# Autodesk Inventor assembly: tandembox_intivo
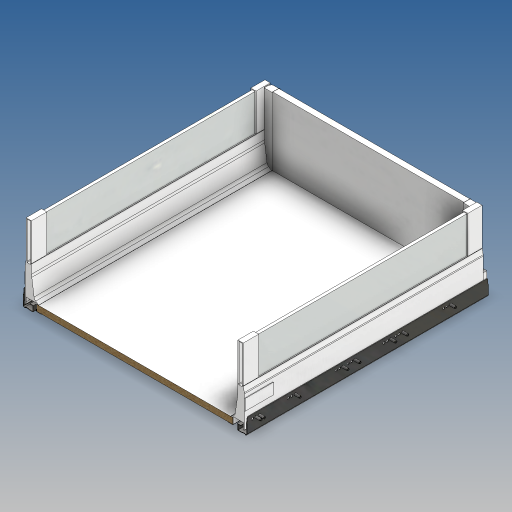
[picture p0: Inventor's stored thumbnail of the model, 512x512]
Saved by Autodesk Inventor 2023 (Build 270158000, 158)
## iProperties
RuleStatus: InUse
Category: Drawer
AfterAnyParamChange0: ConstraintRule
AfterComponentSuppressionChange0: ConstraintRule
Created: 2020-01-10
Part Number: tandembox_intivo
Document SubType Name: Assembly
Designer: RokasM
Author: RokasM
## iProperties of the stored document MemberDocs/xAaaaavdaAaaaaaaaAaaaq5iiOc
Category: Drawer
RuleStatus: InUse
Created: 2020-01-10
Part Number: tandembox_intivo
Document SubType Name: Assembly
Designer: RokasM
AfterAnyParamChange0: ConstraintRule
AfterComponentSuppressionChange0: ConstraintRule
Author: RokasM
## Documents named in this file (41)
- C:\W4INV 2024 Design\iBOX LIBRARY\Drawers\Blum TANDEMBOX\tandembox_intivo.iam
- @tandembox_intivo.iam
- C:\W4INV 2023 Design\iBOX LIBRARY\Drawers\Blum TANDEMBOX\Parts\01_base.ipt
- C:\W4INV 2023 Design\iBOX LIBRARY\Drawers\Blum TANDEMBOX\Parts\02_back.ipt
- C:\W4INV 2023 Design\iBOX LIBRARY\Drawers\Blum TANDEMBOX\Parts\03_drawer_side.ipt
- C:\W4INV 2023 Design\iBOX LIBRARY\Drawers\Blum TANDEMBOX\Parts\04_right_fixing.ipt
- C:\W4INV 2023 Design\iBOX LIBRARY\Drawers\Blum TANDEMBOX\Parts\05_boxcover_front.ipt
- C:\W4INV 2023 Design\iBOX LIBRARY\Drawers\Blum TANDEMBOX\Parts\06_boxcover_back.ipt
- C:\W4INV 2023 Design\iBOX LIBRARY\Drawers\Blum TANDEMBOX\Parts\07_cabinet_profile.ipt
- C:\W4INV 2023 Design\iBOX LIBRARY\Drawers\Blum TANDEMBOX\Parts\08_roller.ipt
- C:\W4INV 2023 Design\iBOX LIBRARY\Drawers\Blum TANDEMBOX\Parts\09_glass.ipt
- C:\W4INV 2023 Design\iBOX LIBRARY\Drawers\Blum TANDEMBOX\Parts\10_hole1.ipt
- C:\W4INV 2023 Design\iBOX LIBRARY\Drawers\Blum TANDEMBOX\Parts\11_hole2.ipt
- C:\W4INV 2023 Design\iBOX LIBRARY\Drawers\Blum TANDEMBOX\Parts\12_hole3.ipt
- C:\W4INV 2023 Design\iBOX LIBRARY\Drawers\Blum TANDEMBOX\Parts\13_hole4.ipt
- C:\W4INV 2023 Design\iBOX LIBRARY\Drawers\Blum TANDEMBOX\Parts\14_hole5.ipt
- C:\W4INV 2023 Design\iBOX LIBRARY\Drawers\Blum TANDEMBOX\Parts\15_hole6.ipt
- C:\W4INV 2023 Design\iBOX LIBRARY\Drawers\Blum TANDEMBOX\Parts\16_hole7.ipt
- C:\W4INV 2023 Design\iBOX LIBRARY\Drawers\Blum TANDEMBOX\Parts\17_screw.ipt
- C:\W4INV 2023 Design\iBOX LIBRARY\Drawers\Blum TANDEMBOX\tandembox_intivo.ipt
- C:\W4INV 2023 Design\iBOX LIBRARY\Drawers\Blum TANDEMBOX\Parts\18_boxcap.ipt
- C:\W4INV 2024 Design\iBOX LIBRARY\Drawers\Blum TANDEMBOX\Parts\01_base.ipt
- C:\W4INV 2024 Design\iBOX LIBRARY\Drawers\Blum TANDEMBOX\Parts\02_back.ipt
- C:\W4INV 2024 Design\iBOX LIBRARY\Drawers\Blum TANDEMBOX\Parts\03_drawer_side.ipt
- C:\W4INV 2024 Design\iBOX LIBRARY\Drawers\Blum TANDEMBOX\Parts\04_right_fixing.ipt
- C:\W4INV 2024 Design\iBOX LIBRARY\Drawers\Blum TANDEMBOX\Parts\05_boxcover_front.ipt
- C:\W4INV 2024 Design\iBOX LIBRARY\Drawers\Blum TANDEMBOX\Parts\06_boxcover_back.ipt
- C:\W4INV 2024 Design\iBOX LIBRARY\Drawers\Blum TANDEMBOX\Parts\07_cabinet_profile.ipt
- C:\W4INV 2024 Design\iBOX LIBRARY\Drawers\Blum TANDEMBOX\Parts\08_roller.ipt
- C:\W4INV 2024 Design\iBOX LIBRARY\Drawers\Blum TANDEMBOX\Parts\09_glass.ipt
- C:\W4INV 2024 Design\iBOX LIBRARY\Drawers\Blum TANDEMBOX\Parts\10_hole1.ipt
- C:\W4INV 2024 Design\iBOX LIBRARY\Drawers\Blum TANDEMBOX\Parts\11_hole2.ipt
- C:\W4INV 2024 Design\iBOX LIBRARY\Drawers\Blum TANDEMBOX\Parts\12_hole3.ipt
- C:\W4INV 2024 Design\iBOX LIBRARY\Drawers\Blum TANDEMBOX\Parts\13_hole4.ipt
- C:\W4INV 2024 Design\iBOX LIBRARY\Drawers\Blum TANDEMBOX\Parts\14_hole5.ipt
- C:\W4INV 2024 Design\iBOX LIBRARY\Drawers\Blum TANDEMBOX\Parts\15_hole6.ipt
- C:\W4INV 2024 Design\iBOX LIBRARY\Drawers\Blum TANDEMBOX\Parts\16_hole7.ipt
- C:\W4INV 2024 Design\iBOX LIBRARY\Drawers\Blum TANDEMBOX\Parts\17_screw.ipt
- C:\W4INV 2024 Design\iBOX LIBRARY\Drawers\Blum TANDEMBOX\tandembox_intivo.ipt
- C:\W4INV 2024 Design\iBOX LIBRARY\Drawers\Blum TANDEMBOX\Parts\18_boxcap.ipt
- C:\W4INV 2023 Design\iBOX LIBRARY\Drawers\Blum TANDEMBOX\tandembox_intivo.iam
## Components (26 placed, 19 different names)
1. @skeleton
2. @01_base:1 — Flush:14, Flush:15, Flush:16
3. @02_back:1 — Flush:9, Flush:10, Flush:11, Flush:23, Flush:24
4. @03_drawer_side:1 — Flush:1, Mate:8, Flush:2, Flush:3, Mate:9, Mate:10, Flush:12, Flush:13, Flush:14, Flush:15, Flush:16, Flush:17, Flush:21, Mate:12, Flush:22
5. @04_right_fixing:1 — Flush:6, Flush:7, Flush:8, Flush:9, Flush:10, Flush:11, Flush:25
6. @05_boxcover_front:1 — Flush:1, Mate:8, Flush:2, Flush:4, Flush:5, Mate:11
7. @06_boxcover_back:1 — Flush:3, Mate:9, Mate:10, Flush:6, Flush:7, Flush:8
8. @07_cabinet_profile:1 — Flush:12, Flush:13, Flush:18, Flush:19, Flush:20, Flush:26, Flush:27, Flush:28, Flush:29, Mate:13, Mate:14, Mate:15, Mate:16, Flush:30, Mate:17
9. @08_roller:1 — Flush:17, Flush:18, Flush:19, Flush:20
10. @09_glass:1 — Flush:4, Flush:5, Mate:11
11. @10_hole1:1
12. @11_hole2:1
13. @12_hole3:1
14. @13_hole4:1
15. @14_hole5:1
16. @15_hole6:1
17. @16_hole7:1
18. @17_screw:1
19. @17_screw:2
20. @17_screw:3
21. @17_screw:4 — Flush:30, Mate:17
22. @17_screw:5 — Flush:26, Mate:13
23. @17_screw:6 — Flush:27, Mate:14
24. @17_screw:7 — Flush:28, Mate:15
25. @17_screw:8 — Flush:29, Mate:16
26. @18_boxcap:1 — Flush:21, Mate:12, Flush:22, Flush:23, Flush:24, Flush:25
## Relationships (40: Flush 30, Mate 10)
- Flush:1: @03_drawer_side:1 ↔ @05_boxcover_front:1
- Mate:8: @03_drawer_side:1 ↔ @05_boxcover_front:1
- Flush:2 (0.45 mm): @03_drawer_side:1 ↔ @05_boxcover_front:1
- Flush:3: @03_drawer_side:1 ↔ @06_boxcover_back:1
- Mate:9: @03_drawer_side:1 ↔ @06_boxcover_back:1
- Mate:10 (-2.4 mm): @03_drawer_side:1 ↔ @06_boxcover_back:1
- Flush:4 (2.7 mm): @05_boxcover_front:1 ↔ @09_glass:1
- Flush:5 (3.1 mm): @05_boxcover_front:1 ↔ @09_glass:1
- Mate:11 (0.3 mm): @05_boxcover_front:1 ↔ @09_glass:1
- Flush:6 (3.8 mm): @04_right_fixing:1 ↔ @06_boxcover_back:1
- Flush:7 (15 mm): @04_right_fixing:1 ↔ @06_boxcover_back:1
- Flush:8 (33.85 mm): @04_right_fixing:1 ↔ @06_boxcover_back:1
- Flush:9: @02_back:1 ↔ @04_right_fixing:1
- Flush:10 (17 mm): @02_back:1 ↔ @04_right_fixing:1
- Flush:11 (0.55 mm): @02_back:1 ↔ @04_right_fixing:1
- Flush:12 (6.2 mm): @03_drawer_side:1 ↔ @07_cabinet_profile:1
- Flush:13 (27.6 mm): @03_drawer_side:1 ↔ @07_cabinet_profile:1
- Flush:14: @01_base:1 ↔ @03_drawer_side:1
- Flush:15 (1 mm): @01_base:1 ↔ @03_drawer_side:1
- Flush:16 (1.5 mm): @01_base:1 ↔ @03_drawer_side:1
- Flush:17 (32 mm): @03_drawer_side:1 ↔ @08_roller:1
- Flush:18 (14.32 mm): @07_cabinet_profile:1 ↔ @08_roller:1
- Flush:19 (21.72 mm): @07_cabinet_profile:1 ↔ @08_roller:1
- Flush:20 (1.8 mm): @07_cabinet_profile:1 ↔ @08_roller:1
- Flush:21: @03_drawer_side:1 ↔ @18_boxcap:1
- Mate:12: @03_drawer_side:1 ↔ @18_boxcap:1
- Flush:22 (0.27 mm): @03_drawer_side:1 ↔ @18_boxcap:1
- Flush:23 (0.5 mm): @02_back:1 ↔ @18_boxcap:1
- Flush:24 (3.8 mm): @02_back:1 ↔ @18_boxcap:1
- Flush:25 (34.65 mm): @04_right_fixing:1 ↔ @18_boxcap:1
- Flush:26 (13.5 mm): @07_cabinet_profile:1 ↔ @17_screw:5
- Flush:27 (13.5 mm): @07_cabinet_profile:1 ↔ @17_screw:6
- Flush:28 (13.5 mm): @07_cabinet_profile:1 ↔ @17_screw:7
- Flush:29 (13.5 mm): @07_cabinet_profile:1 ↔ @17_screw:8
- Mate:13: @07_cabinet_profile:1 ↔ @17_screw:5
- Mate:14: @07_cabinet_profile:1 ↔ @17_screw:6
- Mate:15: @07_cabinet_profile:1 ↔ @17_screw:7
- Mate:16: @07_cabinet_profile:1 ↔ @17_screw:8
- Flush:30 (13.5 mm): @07_cabinet_profile:1 ↔ @17_screw:4
- Mate:17: @07_cabinet_profile:1 ↔ @17_screw:4
## Named parameters: box_depth = 653 mm
